# Autodesk Inventor assembly: two-section-bellows-on-bearings
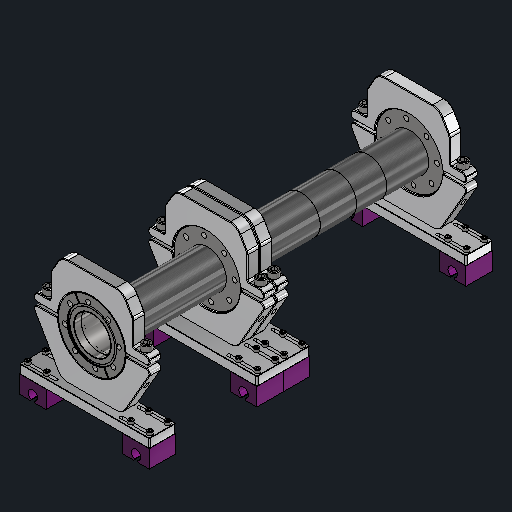
[picture p0: Inventor's stored thumbnail of the model, 512x512]
Saved by Autodesk Inventor 2027.1 (Build 311270010, 270A)
## iProperties
Part Number: two-section-bellows-on-bearings
Document SubType Name: Assembly
Designer: queezz
Author: queezz
## Documents named in this file (8)
- C:\Users\queezz\Dropbox\Drawings\pihti-cad\bellows-probe\two-section-bellows-on-bearings.iam
- C:\Users\queezz\Dropbox\Drawings\pihti-cad\bellows-probe\flange-camp-114.ipt
- C:\Users\queezz\Dropbox\Drawings\pihti-cad\bellows-probe\bellows_flange.ipt
- C:\Users\queezz\Dropbox\Drawings\pihti-cad\bellows-probe\instead-of-bellows.ipt
- C:\Users\queezz\Dropbox\Drawings\pihti-cad\bellows-probe\clamp-foot.ipt
- C:\Users\queezz\Documents\Inventor\Content Center Files\R2027\en-US\AS 1420\AS 1420 - 1973 - M10 x 30.ipt
- C:\Users\queezz\Dropbox\Drawings\pihti-cad\bellows-probe\clamp-foot-double.ipt
- C:\Users\queezz\Dropbox\Drawings\pihti-cad\bellows-probe\linearbearing-bolted.iam
## Components (35 placed, 7 different names)
1. flange-camp-114:1
2. flange-camp-114:2 — Rotational:3
3. bellows_flange:1
4. bellows_flange:2
5. instead-of-bellows:1
6. instead-of-bellows:2
7. clamp-foot:2
8. instead-of-bellows:3
9. instead-of-bellows:4
10. AS 1420 - Metric M10 x 30:1
11. AS 1420 - Metric M10 x 30:2
12. AS 1420 - Metric M10 x 30:3
13. AS 1420 - Metric M10 x 30:4
14. flange-camp-114:3 — Rigid:21
15. flange-camp-114:4
16. bellows_flange:3
17. bellows_flange:4
18. instead-of-bellows:5
19. instead-of-bellows:6
20. clamp-foot:3
21. instead-of-bellows:7
22. instead-of-bellows:8
23. AS 1420 - Metric M10 x 30:5
24. AS 1420 - Metric M10 x 30:6
25. AS 1420 - Metric M10 x 30:7
26. AS 1420 - Metric M10 x 30:8
27. clamp-foot-double:1 — Rotational:3, Rigid:21
28. linearbearing-bolted:7 [sub-assembly]
29. linearbearing-bolted:1 [sub-assembly]
30. linearbearing-bolted:2 [sub-assembly]
31. linearbearing-bolted:3 [sub-assembly]
32. linearbearing-bolted:4 [sub-assembly]
33. linearbearing-bolted:5 [sub-assembly]
34. linearbearing-bolted:6 [sub-assembly]
35. linearbearing-bolted:8 [sub-assembly]
## Relationships (76: Mate 31, Flush 23, WeldJoint 17, Angle 4, RevoluteJoint 1)
- [Mate]: linearbearing-bolted:1 ↔ linearbearing-bolted:8
- [Flush]: flange-camp-114:1 ↔ clamp-foot:2
- [Mate]: flange-camp-114:1 ↔ clamp-foot:2
- [Mate]: flange-camp-114:1 ↔ clamp-foot:2
- [WeldJoint]: flange-camp-114:1 ↔ bellows_flange:2
- [WeldJoint]: flange-camp-114:1 ↔ AS 1420 - Metric M10 x 30:2
- [WeldJoint]: flange-camp-114:1 ↔ AS 1420 - Metric M10 x 30:1
- [Flush]: flange-camp-114:1 ↔ bellows_flange:2
- [Mate]: flange-camp-114:1 ↔ bellows_flange:2
- [Angle] (150 deg): flange-camp-114:1 ↔ bellows_flange:2
- [WeldJoint]: flange-camp-114:2 ↔ bellows_flange:1
- [WeldJoint]: flange-camp-114:2 ↔ AS 1420 - Metric M10 x 30:4
- [WeldJoint]: flange-camp-114:2 ↔ AS 1420 - Metric M10 x 30:3
- [Flush]: flange-camp-114:2 ↔ bellows_flange:1
- [Mate]: flange-camp-114:2 ↔ bellows_flange:1
- [Angle] (30 deg): flange-camp-114:2 ↔ bellows_flange:1
- [WeldJoint]: bellows_flange:1 ↔ instead-of-bellows:2
- [Mate] (-650 mm): bellows_flange:1 ↔ bellows_flange:2
- [WeldJoint]: bellows_flange:2 ↔ instead-of-bellows:1
- [Flush]: linearbearing-bolted:1 ↔ linearbearing-bolted:3
- [Mate]: linearbearing-bolted:1 ↔ linearbearing-bolted:4
- [Flush]: linearbearing-bolted:2 ↔ linearbearing-bolted:4
- [Flush]: linearbearing-bolted:2 ↔ linearbearing-bolted:4
- [Mate]: linearbearing-bolted:2 ↔ linearbearing-bolted:3
- [Flush]: clamp-foot:2 ↔ linearbearing-bolted:2
- [Flush]: clamp-foot:2 ↔ linearbearing-bolted:4
- [Flush]: clamp-foot:2 ↔ linearbearing-bolted:4
- [Flush]: clamp-foot:2 ↔ linearbearing-bolted:4
- [Mate]: instead-of-bellows:1 ↔ instead-of-bellows:2
- [Mate]: instead-of-bellows:1 ↔ instead-of-bellows:4
- [Mate] (-200 mm): instead-of-bellows:1 ↔ instead-of-bellows:4
- [Mate]: instead-of-bellows:2 ↔ instead-of-bellows:3
- [Mate]: instead-of-bellows:2 ↔ instead-of-bellows:3
- [Mate]: instead-of-bellows:3 ↔ instead-of-bellows:4
- [WeldJoint]: flange-camp-114:3 ↔ bellows_flange:4
- [WeldJoint]: flange-camp-114:3 ↔ AS 1420 - Metric M10 x 30:6
- [WeldJoint]: flange-camp-114:3 ↔ AS 1420 - Metric M10 x 30:5
- [Flush]: flange-camp-114:3 ↔ bellows_flange:4
- [Mate]: flange-camp-114:3 ↔ bellows_flange:4
- [Angle] (150 deg): flange-camp-114:3 ↔ bellows_flange:4
- [Mate]: flange-camp-114:4 ↔ clamp-foot:3
- [Mate]: flange-camp-114:4 ↔ clamp-foot:3
- [Flush]: flange-camp-114:4 ↔ clamp-foot:3
- [WeldJoint]: flange-camp-114:4 ↔ bellows_flange:3
- [WeldJoint]: flange-camp-114:4 ↔ AS 1420 - Metric M10 x 30:8
- [WeldJoint]: flange-camp-114:4 ↔ AS 1420 - Metric M10 x 30:7
- [Flush]: flange-camp-114:4 ↔ bellows_flange:3
- [Mate]: flange-camp-114:4 ↔ bellows_flange:3
- [Angle] (30 deg): flange-camp-114:4 ↔ bellows_flange:3
- [WeldJoint]: bellows_flange:3 ↔ instead-of-bellows:6
- [Mate] (-650 mm): bellows_flange:3 ↔ bellows_flange:4
- [WeldJoint]: bellows_flange:4 ↔ instead-of-bellows:5
- [Flush]: linearbearing-bolted:7 ↔ linearbearing-bolted:5
- [Flush]: clamp-foot:3 ↔ linearbearing-bolted:5
- [Mate]: linearbearing-bolted:5 ↔ linearbearing-bolted:8
- [Flush]: clamp-foot:3 ↔ linearbearing-bolted:5
- [Flush]: linearbearing-bolted:6 ↔ linearbearing-bolted:8
- [Flush]: linearbearing-bolted:6 ↔ linearbearing-bolted:8
- [Mate]: linearbearing-bolted:7 ↔ linearbearing-bolted:6
- [Mate]: clamp-foot:3 ↔ linearbearing-bolted:7
- [Flush]: clamp-foot:3 ↔ linearbearing-bolted:7
- [Flush]: clamp-foot:3 ↔ linearbearing-bolted:7
- [Mate]: instead-of-bellows:5 ↔ instead-of-bellows:6
- [Mate]: instead-of-bellows:5 ↔ instead-of-bellows:8
- [Mate] (-200 mm): instead-of-bellows:5 ↔ instead-of-bellows:8
- [Mate]: instead-of-bellows:6 ↔ instead-of-bellows:7
- [Mate]: instead-of-bellows:6 ↔ instead-of-bellows:7
- [Mate]: instead-of-bellows:7 ↔ instead-of-bellows:8
- [Mate]: linearbearing-bolted:3 ↔ linearbearing-bolted:6
- [Mate]: clamp-foot-double:1 ↔ linearbearing-bolted:8
- [Mate]: clamp-foot:2 ↔ linearbearing-bolted:4
- Rotational:3 [RevoluteJoint]: flange-camp-114:2 ↔ clamp-foot-double:1
- Rigid:21 [WeldJoint]: flange-camp-114:3 ↔ clamp-foot-double:1
- [Flush]: clamp-foot-double:1 ↔ linearbearing-bolted:1
- [Flush]: clamp-foot-double:1 ↔ linearbearing-bolted:3
- [Flush]: clamp-foot-double:1 ↔ linearbearing-bolted:6
## Named parameters: d53_d56 = 0 mm, d79_d113 = 0 mm, d80_d114 = 0 mm, d81_d55 = 0 mm, d82_d67 = 0 mm, d83_d68 = 150 deg, d84_d109 = 0 mm, d87_d111 = 0 mm, d88_d112 = 0 mm, d89_d69 = 0 mm, d90_d70 = 0 mm, d95_d75 = 30 deg, d96_d110 = 0 mm, d98_d71 = 0 mm, d99_d72 = 0 mm, d100_d73 = 0 mm, d101_d40 = -650 mm, d102_d41 = -135 mm, d103_d42 = -485 mm, d104_d22 = 0 mm, d105_d21 = 0 mm, d106_d36 = 0 mm, d107_d45 = 0 mm, d108_d74 = 0 mm, d115_d18 = 0 mm, d116_d37 = 0 mm, d118_d17 = 0 mm, d119_d19 = 0 mm, d126_d91 = 0 mm, d127_d24_d26 = 0 mm, d132_d61 = -200 mm, d133_d62 = 0 mm, d134_d63 = -200 mm, d135_d23 = 0 mm, d136_d57 = 0 mm, d137_d58 = 0 mm, d138_d59 = 0 mm, d139_d60 = -200 mm, d140_d64 = 0 mm, d141_d65 = 0 mm, d142_d66 = -200 mm
